# Autodesk Inventor assembly: CNC Plotter
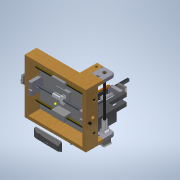
[picture p0: Inventor's stored thumbnail of the model, 180x180]
Saved by Autodesk Inventor 2021.3 (Build 253353000, 353)
## iProperties
Created: 2021-06-01
Part Number: CNC Plotter
Document SubType Name: Assembly
Designer: vivek
Author: vivek
## Documents named in this file (19)
- C:\Users\vivek\OneDrive\Documents\II Sem\EE\Pattern Drawing Bot\Final3DModel\Plotter_Assembled.iam
- C:\Users\vivek\OneDrive\Documents\II Sem\EE\Pattern Drawing Bot\Final3DModel\Holder.ipt
- C:\Users\vivek\OneDrive\Documents\II Sem\EE\Pattern Drawing Bot\Final3DModel\Rotator.ipt
- C:\Users\vivek\OneDrive\Documents\II Sem\EE\Pattern Drawing Bot\Final3DModel\Rod.ipt
- C:\Users\vivek\OneDrive\Documents\II Sem\EE\Pattern Drawing Bot\Final3DModel\Plate.ipt
- C:\Users\vivek\OneDrive\Documents\II Sem\EE\Pattern Drawing Bot\Final3DModel\Base.ipt
- C:\Users\vivek\OneDrive\Documents\II Sem\EE\Pattern Drawing Bot\Final3DModel\Bottom_Mover.ipt
- C:\Users\vivek\OneDrive\Documents\II Sem\EE\Pattern Drawing Bot\Final3DModel\Stepper Motor NEMA 17.ipt
- C:\Users\vivek\OneDrive\Documents\II Sem\EE\Pattern Drawing Bot\Final3DModel\Support.ipt
- C:\Users\vivek\OneDrive\Documents\II Sem\EE\Pattern Drawing Bot\Final3DModel\Pen_Mover.ipt
- C:\Users\vivek\OneDrive\Documents\II Sem\EE\Pattern Drawing Bot\Final3DModel\Pen_Holder.ipt
- C:\Users\vivek\OneDrive\Documents\II Sem\EE\Pattern Drawing Bot\Final3DModel\Stand.ipt
- C:\Users\vivek\OneDrive\Documents\II Sem\EE\Pattern Drawing Bot\Final3DModel\Pen.ipt
- C:\Users\vivek\OneDrive\Documents\II Sem\EE\Pattern Drawing Bot\Final3DModel\remote\remote.iam
- C:\Users\vivek\OneDrive\Documents\II Sem\EE\Pattern Drawing Bot\Final3DModel\buzzer.ipt
- C:\Users\vivek\OneDrive\Documents\II Sem\EE\Pattern Drawing Bot\Final3DModel\gm spinac tlacitkovy BB15AH-FA.ipt
- C:\Users\vivek\OneDrive\Documents\II Sem\EE\Pattern Drawing Bot\Final3DModel\L-1503CB 1GD.ipt
- C:\Users\vivek\OneDrive\Documents\II Sem\EE\Pattern Drawing Bot\Final3DModel\L-1503CB 1ID.ipt
- C:\Users\vivek\OneDrive\Documents\II Sem\EE\Pattern Drawing Bot\Final3DModel\IR.ipt
## Components (30 placed, 18 different names)
1. Holder:1 — Mate:1, Flush:1, Mate:5, Mate:12, Mate:16, Flush:11, Mate:17
2. Rotator:1 — Mate:2, Mate:12, Mate:13, Flush:9
3. Rod:1 — Mate:1, Flush:1, Mate:2, Mate:3, Flush:2
4. Holder:2 — Mate:3, Flush:2, Mate:15
5. Plate:1 — Mate:5, Mate:11, Mate:13, Flush:9, Mate:15
6. Holder:3 — Flush:6, Flush:26
7. Rotator:2 — Mate:27, Mate:28, Flush:17
8. Rod:2 — Mate:24
9. Holder:4 — Flush:6, Mate:11, Mate:21, Mate:25, Mate:27
10. Base:1 — Mate:16, Flush:11, Mate:17, Mate:19, Flush:13, Mate:20, Flush:14, Mate:21, Mate:22, Mate:23, Flush:16, Flush:26, Mate:46, Mate:47, Mate:49
11. Bottom_Mover:1 — Mate:19, Flush:13
12. Bottom_Mover:2 — Mate:20, Flush:14
13. Stepper Motor NEMA 17:1 — Mate:22, Mate:23
14. Stepper Motor NEMA 17:2 — Mate:24, Mate:25
15. Rod:3 — Flush:16, Mate:32, Mate:48, Mate:49, Insert:1
16. Support:1 — Mate:28, Flush:17, Mate:32, Mate:33, Flush:18, Flush:19, Mate:35, Flush:20, Flush:21, Mate:48, Insert:1
17. Stepper Motor NEMA 17:3 — Mate:36, Mate:38
18. Holder:5 — Mate:35, Flush:20, Flush:21, Flush:22, Mate:40, Flush:23, Mate:43
19. Holder:6 — Mate:33, Flush:18, Flush:19, Mate:36, Mate:37, Mate:38
20. Pen_Mover:1 — Mate:37, Flush:22, Mate:39, Insert:2
21. Rotator:3 — Mate:39, Mate:40, Mate:44, Flush:24, Insert:2
22. Pen_Holder:1 — Mate:41, Mate:42, Flush:24, Flush:25, Tangent:1
23. Stand:1 — Mate:41, Mate:42, Flush:23, Mate:43, Mate:44, Mate:45
24. Pen:1 — Flush:25, Tangent:1, Mate:45
25. remote:1 [sub-assembly]
26. buzzer:1 — Mate:46
27. gm spinac tlacitkovy BB15AH-FA:1 — Mate:47
28. L-1503CB 1GD:1
29. L-1503CB 1ID:1
30. IR:1
## Relationships (62: Mate 39, Flush 20, Insert 2, Tangent 1)
- Mate:1: Holder:1 ↔ Rod:1
- Flush:1: Holder:1 ↔ Rod:1
- Mate:2: Rotator:1 ↔ Rod:1
- Mate:3: Rod:1 ↔ Holder:2
- Flush:2: Rod:1 ↔ Holder:2
- Mate:5: Holder:1 ↔ Plate:1
- [Mate]: Holder:3 ↔ Rod:2
- [Flush]: Holder:3 ↔ Rod:2
- [Mate]: Rotator:2 ↔ Rod:2
- [Mate]: Rod:2 ↔ Holder:4
- [Flush]: Rod:2 ↔ Holder:4
- Flush:6: Holder:3 ↔ Holder:4
- Mate:11: Plate:1 ↔ Holder:4
- Mate:12: Holder:1 ↔ Rotator:1
- Mate:13: Rotator:1 ↔ Plate:1
- Flush:9: Rotator:1 ↔ Plate:1
- Mate:15: Holder:2 ↔ Plate:1
- Mate:16: Holder:1 ↔ Base:1
- Flush:11: Holder:1 ↔ Base:1
- Mate:17: Holder:1 ↔ Base:1
- Mate:19: Base:1 ↔ Bottom_Mover:1
- Flush:13: Base:1 ↔ Bottom_Mover:1
- Mate:20: Base:1 ↔ Bottom_Mover:2
- Flush:14: Base:1 ↔ Bottom_Mover:2
- Mate:21: Holder:4 ↔ Base:1
- Mate:22: Base:1 ↔ Stepper Motor NEMA 17:1
- Mate:23: Base:1 ↔ Stepper Motor NEMA 17:1
- Mate:24: Rod:2 ↔ Stepper Motor NEMA 17:2
- Mate:25: Holder:4 ↔ Stepper Motor NEMA 17:2
- Flush:16: Base:1 ↔ Rod:3
- Mate:27: Rotator:2 ↔ Holder:4
- Mate:28: Rotator:2 ↔ Support:1
- Flush:17: Rotator:2 ↔ Support:1
- Mate:32: Rod:3 ↔ Support:1
- Mate:33: Support:1 ↔ Holder:6
- Flush:18: Support:1 ↔ Holder:6
- Flush:19: Support:1 ↔ Holder:6
- Mate:35: Support:1 ↔ Holder:5
- Flush:20: Support:1 ↔ Holder:5
- Flush:21: Support:1 ↔ Holder:5
- Mate:36: Stepper Motor NEMA 17:3 ↔ Holder:6
- Mate:37: Holder:6 ↔ Pen_Mover:1
- Flush:22: Holder:5 ↔ Pen_Mover:1
- Mate:38: Stepper Motor NEMA 17:3 ↔ Holder:6
- Mate:39: Pen_Mover:1 ↔ Rotator:3
- Mate:40: Holder:5 ↔ Rotator:3
- Mate:41: Pen_Holder:1 ↔ Stand:1
- Mate:42: Pen_Holder:1 ↔ Stand:1
- Flush:23: Holder:5 ↔ Stand:1
- Mate:43: Holder:5 ↔ Stand:1
- Mate:44: Rotator:3 ↔ Stand:1
- Flush:24: Rotator:3 ↔ Pen_Holder:1
- Flush:25 (-50 mm): Pen_Holder:1 ↔ Pen:1
- Tangent:1: Pen_Holder:1 ↔ Pen:1
- Mate:45: Stand:1 ↔ Pen:1
- Flush:26: Holder:3 ↔ Base:1
- Mate:46: Base:1 ↔ buzzer:1
- Mate:47 (5.062 mm): Base:1 ↔ gm spinac tlacitkovy BB15AH-FA:1
- Mate:48: Rod:3 ↔ Support:1
- Mate:49: Base:1 ↔ Rod:3
- Insert:1 (-215 mm): Rod:3 ↔ Support:1
- Insert:2 (20 mm): Pen_Mover:1 ↔ Rotator:3
## Named parameters: d9_d2 = 0 mm, d10_d3 = 0 mm, d11_d4 = 0 mm, d12_d0 = 0 mm, d13_d1 = 0 mm
